# Autodesk Inventor assembly: compdispenses
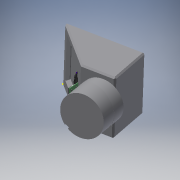
[picture p0: Inventor's stored thumbnail of the model, 180x180]
Saved by Autodesk Inventor 2019 (Build 230136000, 136)
## iProperties
Created: 2020-02-26
Part Number: compdispenses
Document SubType Name: Assembly
Designer: hp
Author: hp
## Documents named in this file (7)
- D:\engineering exploration\reveiw\compdispenses.iam
- D:\engineering exploration\reveiw\dc.ipt
- D:\engineering exploration\reveiw\final dispenser.ipt
- D:\engineering exploration\reveiw\LCDmodule.ipt
- D:\engineering exploration\reveiw\scanner3dmodel.ipt
- D:\engineering exploration\reveiw\keyboard_kb1604pnb_65x64x8-9.ipt
- D:\engineering exploration\reveiw\covering unit.ipt
## Components (6 placed, 6 different names)
1. final dispenser:1 — Mate:1, Mate:2, Mate:3, Mate:4, Mate:5, Mate:6
2. dc:1 — Mate:1, Mate:2, Mate:3, Mate:4, Mate:5
3. LCDmodule:1
4. scanner3dmodel:1
5. keyboard_kb1604pnb_65x64x8-9:1
6. covering unit:1 — Mate:6
## Relationships (6: Mate 6)
- Mate:1: final dispenser:1 ↔ dc:1
- Mate:2: final dispenser:1 ↔ dc:1
- Mate:3: final dispenser:1 ↔ dc:1
- Mate:4: final dispenser:1 ↔ dc:1
- Mate:5: final dispenser:1 ↔ dc:1
- Mate:6: final dispenser:1 ↔ covering unit:1
